# Autodesk Inventor assembly: GE-12016
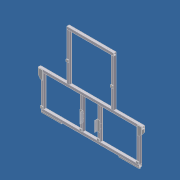
[picture p0: Inventor's stored thumbnail of the model, 180x180]
Saved by Autodesk Inventor 2012 (Build 160160000, 160)
## iProperties
Created: 2011-06-01
Part Number: GE-12016
Document SubType Name: Assembly
Designer: dfoster
Description: Backboard Frame
Title: Backboard Frame
Author: dfoster
## Documents named in this file (9)
- C:\Data Folder\FRC 2012 Field\Components\GE-12016.iam
- C:\Data Folder\FRC 2012 Field\Components\GE-12016-01.ipt
- C:\Data Folder\FRC 2012 Field\Components\GE-12016-02.ipt
- C:\Data Folder\FRC 2012 Field\Components\GE-12016-03.ipt
- C:\Data Folder\FRC 2012 Field\Components\GE-12016-05.ipt
- C:\Data Folder\FRC 2012 Field\Components\GE-12016-04.ipt
- C:\Data Folder\FRC 2012 Field\Components\GE-12016-06.ipt
- C:\Data Folder\FRC 2012 Field\Components\GE-12016-07.ipt
- C:\Data Folder\FRC 2012 Field\Components\GE-12016-08.ipt
## Components (23 placed, 8 different names)
1. GE-12016-01:2 — Flush:3, Flush:4, Flush:15, Flush:16, Flush:17, Mate:7, Flush:18, Mate:16, Flush:35
2. GE-12016-03:1 — Mate:5, Flush:10, Flush:12, Flush:13, Flush:20, Mate:9
3. GE-12016-03:2 — Flush:11, Flush:21, Mate:8
4. GE-12016-01:1 — Mate:1, Flush:1, Flush:2, Flush:3, Flush:4, Flush:13, Flush:14, Mate:6, Flush:19, Mate:17, Flush:36, Flush:41
5. GE-12016-03:3 — Mate:5, Flush:10, Flush:11, Flush:12, Flush:21, Mate:8, Flush:30, Flush:31, Flush:32, Mate:14, Mate:15, Flush:33, Flush:34
6. GE-12016-02:2 — Flush:14, Mate:6, Flush:15, Flush:16, Flush:19, Flush:37, Flush:38, Mate:18, Mate:19, Flush:39, Flush:40, Flush:44, Flush:45, Mate:25, Flush:50, Flush:51, Mate:26, Flush:52, Flush:53
7. GE-12016-05:1 — Flush:17, Mate:7, Flush:18, Flush:20, Mate:9, Mate:10, Mate:11, Flush:22, Flush:23, Mate:12, Mate:13, Flush:26, Flush:27, Flush:28, Flush:49
8. GE-12016-04:1 — Mate:10, Flush:22, Flush:23, Flush:24, Flush:25
9. GE-12016-04:2 — Mate:11, Flush:24, Flush:25
10. GE-12016-04:3 — Mate:13, Flush:27, Flush:28, Flush:29
11. GE-12016-06:1 — Flush:30, Flush:31, Flush:32, Mate:14
12. GE-12016-04:4 — Mate:12, Flush:26, Flush:29
13. GE-12016-06:2 — Mate:15, Flush:33, Flush:34
14. GE-12016-06:6 — Mate:16, Flush:35, Flush:38
15. GE-12016-01:3 — Mate:18, Flush:40, Mate:20, Flush:41, Mate:21, Flush:42, Mate:24, Flush:46
16. GE-12016-01:4 — Mate:19, Flush:39, Mate:20, Mate:22, Flush:43, Mate:23, Flush:47
17. GE-12016-06:5 — Mate:17, Flush:36, Flush:37
18. GE-12016-06:7 — Mate:21, Flush:42, Flush:44
19. GE-12016-06:8 — Mate:22, Flush:43, Flush:45
20. GE-12016-07:1 — Mate:24, Flush:46, Flush:48, Flush:49
21. GE-12016-07:2 — Mate:23, Flush:47, Flush:48
22. GE-12016-08:1 — Mate:26, Flush:52, Flush:53
23. GE-12016-08:2 — Mate:25, Flush:50, Flush:51
## Relationships (71: Flush 48, Mate 23)
- Mate:1: GE-12016-01:1
- Flush:1: GE-12016-01:1
- Flush:2: GE-12016-01:1
- Flush:3: GE-12016-01:2 ↔ GE-12016-01:1
- Flush:4: GE-12016-01:2 ↔ GE-12016-01:1
- Mate:5: GE-12016-03:1 ↔ GE-12016-03:3
- Flush:10: GE-12016-03:1 ↔ GE-12016-03:3
- Flush:11: GE-12016-03:2 ↔ GE-12016-03:3
- Flush:12: GE-12016-03:1 ↔ GE-12016-03:3
- Flush:13 (444.5 mm): GE-12016-03:1 ↔ GE-12016-01:1
- Flush:14: GE-12016-01:1 ↔ GE-12016-02:2
- Mate:6: GE-12016-01:1 ↔ GE-12016-02:2
- Flush:15: GE-12016-01:2 ↔ GE-12016-02:2
- Flush:16: GE-12016-01:2 ↔ GE-12016-02:2
- Flush:17: GE-12016-01:2 ↔ GE-12016-05:1
- Mate:7: GE-12016-01:2 ↔ GE-12016-05:1
- Flush:18 (50.8 mm): GE-12016-01:2 ↔ GE-12016-05:1
- Flush:19: GE-12016-01:1 ↔ GE-12016-02:2
- Flush:20: GE-12016-03:1 ↔ GE-12016-05:1
- Flush:21: GE-12016-03:2 ↔ GE-12016-03:3
- Mate:8: GE-12016-03:2 ↔ GE-12016-03:3
- Mate:9: GE-12016-03:1 ↔ GE-12016-05:1
- Mate:10: GE-12016-05:1 ↔ GE-12016-04:1
- Mate:11: GE-12016-05:1 ↔ GE-12016-04:2
- Flush:22 (-6.35 mm): GE-12016-05:1 ↔ GE-12016-04:1
- Flush:23 (-6.35 mm): GE-12016-05:1 ↔ GE-12016-04:1
- Flush:24: GE-12016-04:1 ↔ GE-12016-04:2
- Flush:25: GE-12016-04:1 ↔ GE-12016-04:2
- Mate:12: GE-12016-05:1 ↔ GE-12016-04:4
- Mate:13: GE-12016-05:1 ↔ GE-12016-04:3
- Flush:26 (6.35 mm): GE-12016-05:1 ↔ GE-12016-04:4
- Flush:27 (-6.35 mm): GE-12016-05:1 ↔ GE-12016-04:3
- Flush:28 (6.35 mm): GE-12016-05:1 ↔ GE-12016-04:3
- Flush:29: GE-12016-04:3 ↔ GE-12016-04:4
- Flush:30: GE-12016-03:3 ↔ GE-12016-06:1
- Flush:31 (3.175 mm): GE-12016-03:3 ↔ GE-12016-06:1
- Flush:32 (482.6 mm): GE-12016-03:3 ↔ GE-12016-06:1
- Mate:14: GE-12016-03:3 ↔ GE-12016-06:1
- Mate:15: GE-12016-03:3 ↔ GE-12016-06:2
- Flush:33 (482.6 mm): GE-12016-03:3 ↔ GE-12016-06:2
- Flush:34 (3.175 mm): GE-12016-03:3 ↔ GE-12016-06:2
- Mate:16: GE-12016-01:2 ↔ GE-12016-06:6
- Flush:35 (3.175 mm): GE-12016-01:2 ↔ GE-12016-06:6
- Mate:17: GE-12016-01:1 ↔ GE-12016-06:5
- Flush:36 (3.175 mm): GE-12016-01:1 ↔ GE-12016-06:5
- Flush:37 (-50.8 mm): GE-12016-02:2 ↔ GE-12016-06:5
- Flush:38 (-50.8 mm): GE-12016-02:2 ↔ GE-12016-06:6
- Mate:18: GE-12016-02:2 ↔ GE-12016-01:3
- Mate:19: GE-12016-02:2 ↔ GE-12016-01:4
- Flush:39: GE-12016-02:2 ↔ GE-12016-01:4
- Flush:40: GE-12016-02:2 ↔ GE-12016-01:3
- Mate:20 (260.35 mm): GE-12016-01:3 ↔ GE-12016-01:4
- Flush:41 (676.275 mm): GE-12016-01:1 ↔ GE-12016-01:3
- Mate:21: GE-12016-01:3 ↔ GE-12016-06:7
- Flush:42 (3.175 mm): GE-12016-01:3 ↔ GE-12016-06:7
- Mate:22: GE-12016-01:4 ↔ GE-12016-06:8
- Flush:43 (3.175 mm): GE-12016-01:4 ↔ GE-12016-06:8
- Flush:44 (50.8 mm): GE-12016-02:2 ↔ GE-12016-06:7
- Flush:45 (50.8 mm): GE-12016-02:2 ↔ GE-12016-06:8
- Mate:23: GE-12016-01:4 ↔ GE-12016-07:2
- Mate:24: GE-12016-01:3 ↔ GE-12016-07:1
- Flush:46 (-6.35 mm): GE-12016-01:3 ↔ GE-12016-07:1
- Flush:47 (-6.35 mm): GE-12016-01:4 ↔ GE-12016-07:2
- Flush:48: GE-12016-07:1 ↔ GE-12016-07:2
- Flush:49 (-266.7 mm): GE-12016-05:1 ↔ GE-12016-07:1
- Mate:25: GE-12016-02:2 ↔ GE-12016-08:2
- Flush:50: GE-12016-02:2 ↔ GE-12016-08:2
- Flush:51: GE-12016-02:2 ↔ GE-12016-08:2
- Mate:26: GE-12016-02:2 ↔ GE-12016-08:1
- Flush:52: GE-12016-02:2 ↔ GE-12016-08:1
- Flush:53: GE-12016-02:2 ↔ GE-12016-08:1
